# Autodesk Inventor assembly: shooter
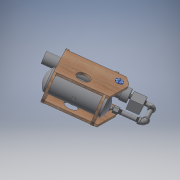
[picture p0: Inventor's stored thumbnail of the model, 180x180]
Saved by Autodesk Inventor 2018 (Build 220112000, 112)
## iProperties
Created: 2017-05-02
Part Number: shooter
Document SubType Name: Assembly
Designer: gsegs
Author: gsegs
## Documents named in this file (11)
- C:\Users\gsegs\OneDrive\Documents\GitHub\RoboEaglesCad2018\shooter.iam
- C:\Users\gsegs\OneDrive\Documents\GitHub\RoboEaglesCad2018\6in pipe.ipt
- C:\Users\gsegs\OneDrive\Documents\GitHub\RoboEaglesCad2018\90 angle pipe.ipt
- C:\Users\gsegs\OneDrive\Documents\GitHub\RoboEaglesCad2018\90 angle pipe 2.ipt
- C:\Users\gsegs\OneDrive\Documents\GitHub\RoboEaglesCad2018\adapter.ipt
- C:\Users\gsegs\OneDrive\Documents\GitHub\RoboEaglesCad2018\long pipe.ipt
- C:\Users\gsegs\OneDrive\Documents\GitHub\RoboEaglesCad2018\air canister.ipt
- C:\Users\gsegs\OneDrive\Documents\GitHub\RoboEaglesCad2018\cannon support front.ipt
- C:\Users\gsegs\OneDrive\Documents\GitHub\RoboEaglesCad2018\solenoid.ipt
- C:\Users\gsegs\OneDrive\Documents\GitHub\RoboEaglesCad2018\cannonSideWall.ipt
- C:\Users\gsegs\OneDrive\Documents\GitHub\RoboEaglesCad2018\am-0096a+500+Hex+Hub+r2.ipt
## Components (16 placed, 10 different names)
1. 6in pipe:1 — Mate:5, Mate:6, Mate:9
2. 6in pipe:2 — Mate:1, Mate:2, Mate:10
3. 90 angle pipe:1 — Mate:2, Mate:4, Mate:5, Mate:10
4. 90 angle pipe 2:1 — Mate:1, Mate:7, Mate:8
5. adapter:1 — Mate:4, Mate:6, Mate:9, Mate:11, Mate:12
6. long pipe:1 — Mate:7, Mate:8, Angle:1, Mate:18, Flush:5, Tangent:1, Tangent:2, Mate:22
7. air canister:1 — Mate:11, Angle:1, Mate:12, Mate:17, Tangent:3, Mate:21, Tangent:4, Angle:4
8. cannon support front:3 — Mate:18, Flush:3, Flush:4, Mate:19, Flush:9, Flush:10
9. cannon support front:4 — Mate:17, Flush:3, Flush:4, Mate:19, Tangent:3, Mate:24, Mate:25
10. solenoid:1 — Flush:5, Tangent:1, Tangent:2
11. cannon support front:5 — Tangent:4
12. cannon support front:6 — Mate:21, Mate:22, Angle:4
13. cannonSideWall:1 — Flush:9, Flush:10, Mate:26, Mate:28
14. cannonSideWall:2 — Mate:24, Mate:25, Mate:27, Mate:29, Angle:3
15. am-0096a+500+Hex+Hub+r2:1 — Mate:26, Mate:28, Angle:2
16. am-0096a+500+Hex+Hub+r2:2 — Mate:27, Mate:29, Angle:2, Angle:3
## Relationships (40: Mate 23, Flush 9, Angle 4, Tangent 4)
- Mate:1: 6in pipe:2 ↔ 90 angle pipe 2:1
- Mate:2: 6in pipe:2 ↔ 90 angle pipe:1
- Mate:4 (134.9375 mm): 90 angle pipe:1 ↔ adapter:1
- Mate:5: 6in pipe:1 ↔ 90 angle pipe:1
- Mate:6: 6in pipe:1 ↔ adapter:1
- Mate:7 (114.3 mm): 90 angle pipe 2:1 ↔ long pipe:1
- Mate:8: 90 angle pipe 2:1 ↔ long pipe:1
- Mate:9 (25.4 mm): 6in pipe:1 ↔ adapter:1
- Mate:10 (12.7 mm): 6in pipe:2 ↔ 90 angle pipe:1
- Mate:11 (8.89 mm): adapter:1 ↔ air canister:1
- Angle:1 (0 deg): long pipe:1 ↔ air canister:1
- Mate:12: adapter:1 ↔ air canister:1
- [Flush]: cannon support front:3 ↔ cannon support front:4
- Mate:17: air canister:1 ↔ cannon support front:4
- Mate:18: long pipe:1 ↔ cannon support front:3
- Flush:3: cannon support front:3 ↔ cannon support front:4
- Flush:4: cannon support front:3 ↔ cannon support front:4
- Flush:5: long pipe:1 ↔ solenoid:1
- Tangent:1 (4 mm): long pipe:1 ↔ solenoid:1
- Tangent:2 (25.4 mm): long pipe:1 ↔ solenoid:1
- Mate:19: cannon support front:3 ↔ cannon support front:4
- Tangent:3 (-196.85 mm): air canister:1 ↔ cannon support front:4
- [Flush]: cannon support front:5 ↔ cannon support front:6
- [Flush]: cannon support front:5 ↔ cannon support front:6
- [Flush]: cannon support front:5 ↔ cannon support front:6
- [Mate]: cannon support front:5 ↔ cannon support front:6
- Mate:21: air canister:1 ↔ cannon support front:6
- Mate:22: long pipe:1 ↔ cannon support front:6
- Tangent:4 (-196.85 mm): air canister:1 ↔ cannon support front:5
- Flush:9: cannon support front:3 ↔ cannonSideWall:1
- Flush:10: cannon support front:3 ↔ cannonSideWall:1
- Mate:24: cannon support front:4 ↔ cannonSideWall:2
- Mate:25: cannon support front:4 ↔ cannonSideWall:2
- Mate:26: cannonSideWall:1 ↔ am-0096a+500+Hex+Hub+r2:1
- Mate:27: cannonSideWall:2 ↔ am-0096a+500+Hex+Hub+r2:2
- Mate:28: cannonSideWall:1 ↔ am-0096a+500+Hex+Hub+r2:1
- Mate:29: cannonSideWall:2 ↔ am-0096a+500+Hex+Hub+r2:2
- Angle:2 (0 deg): am-0096a+500+Hex+Hub+r2:1 ↔ am-0096a+500+Hex+Hub+r2:2
- Angle:3 (0 deg): cannonSideWall:2 ↔ am-0096a+500+Hex+Hub+r2:2
- Angle:4 (0 deg): air canister:1 ↔ cannon support front:6
## Named parameters: d18_d17 = 0 mm, d28_d26 = 0 mm, d29_d18_d17 = 0 mm, d30_d21 = 0 mm, d31_d22 = 0 mm
